# Autodesk Inventor assembly: CARRO
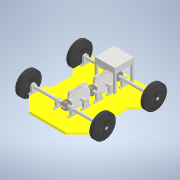
[picture p0: Inventor's stored thumbnail of the model, 180x180]
Saved by Autodesk Inventor 2021 (Build 250183000, 183)
## iProperties
Created: 2021-02-07
Part Number: CARRO
Document SubType Name: Assembly
Designer: rotje
Author: rotje
## Documents named in this file (6)
- C:\Users\rotje\Documents\Inventor\MSF\CARRO.iam
- C:\Users\rotje\Documents\Inventor\MSF\Base-soporte.iam
- C:\Users\rotje\Documents\Inventor\MSF\Eje-engrane.iam
- C:\Users\rotje\Documents\Inventor\MSF\Eje-engrane_chico.iam
- C:\Users\rotje\Documents\Inventor\MSF\Eje_Engrane-llanta.iam
- C:\Users\rotje\Documents\Inventor\MSF\Base_carga.ipt
## Components (7 placed, 5 different names)
1. Base-soporte:1 [sub-assembly] — Insertar:1, Insertar:2, Insertar:3, Coincidencia:1, Coincidencia:2, Coincidencia:3, Coincidencia:4, Coincidencia:5, Coincidencia:6, Coincidencia:7, Coincidencia:8
2. Eje-engrane:1 [sub-assembly] — Insertar:3, Nivelación:1
3. Eje-engrane:2 [sub-assembly] — Insertar:1, Nivelación:2
4. Eje-engrane_chico:1 [sub-assembly] — Insertar:2
5. Eje_Engrane-llanta:1 [sub-assembly] — Nivelación:1, Coincidencia:2
6. Eje_Engrane-llanta:2 [sub-assembly] — Nivelación:2, Coincidencia:3
7. Base_carga:1 — Coincidencia:6, Coincidencia:7, Coincidencia:8
## Relationships (13: Mate 8, Insert 3, Flush 2)
- Insertar:1: Base-soporte:1 ↔ Eje-engrane:2
- Insertar:2: Base-soporte:1 ↔ Eje-engrane_chico:1
- Insertar:3: Base-soporte:1 ↔ Eje-engrane:1
- Coincidencia:1 [Mate]: Base-soporte:1
- Nivelación:1 [Flush]: Eje-engrane:1 ↔ Eje_Engrane-llanta:1
- Nivelación:2 [Flush]: Eje-engrane:2 ↔ Eje_Engrane-llanta:2
- Coincidencia:2 [Mate]: Base-soporte:1 ↔ Eje_Engrane-llanta:1
- Coincidencia:3 [Mate]: Base-soporte:1 ↔ Eje_Engrane-llanta:2
- Coincidencia:4 [Mate]: Base-soporte:1
- Coincidencia:5 [Mate]: Base-soporte:1
- Coincidencia:6 [Mate]: Base-soporte:1 ↔ Base_carga:1
- Coincidencia:7 [Mate]: Base-soporte:1 ↔ Base_carga:1
- Coincidencia:8 [Mate]: Base-soporte:1 ↔ Base_carga:1
